# Autodesk Inventor assembly: illuminationAxis
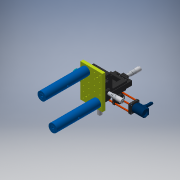
[picture p0: Inventor's stored thumbnail of the model, 180x180]
Saved by Autodesk Inventor 2016 (Build 200138000, 138)
## iProperties
Created: 2016-02-18
Part Number: illuminationAxis
Document SubType Name: Assembly
Designer: sims01
Author: sims01
## Documents named in this file (13)
- H:\Documents\LSFM_3\setup\mechanical\design\lsfm3_mechDesign\illuminationAxis.iam
- H:\Documents\LSFM_3\setup\mechanical\design\lsfm3_mechDesign\thorlabs100150mm2breadboard.ipt
- H:\Documents\LSFM_3\setup\mechanical\design\lsfm3_mechDesign\30mmCageMountingBase.ipt
- H:\Documents\LSFM_3\setup\mechanical\design\lsfm3_mechDesign\sm1CageMount.ipt
- H:\Documents\LSFM_3\setup\mechanical\design\lsfm3_mechDesign\m26sm1ThreadAdapter.ipt
- H:\Documents\LSFM_3\setup\mechanical\design\lsfm3_mechDesign\10X_mitutoyoObj.ipt
- H:\Documents\LSFM_3\setup\mechanical\design\lsfm3_mechDesign\30mmCageRotationMount.ipt
- H:\Documents\LSFM_3\setup\mechanical\design\lsfm3_mechDesign\75mmCylLens.ipt
- H:\Documents\LSFM_3\setup\mechanical\design\lsfm3_mechDesign\12mmFibreCollimator.ipt
- H:\Documents\LSFM_3\setup\mechanical\design\lsfm3_mechDesign\203mmCageRods.ipt
- H:\Documents\LSFM_3\setup\mechanical\design\lsfm3_mechDesign\graduatedIris.ipt
- H:\Documents\LSFM_3\setup\mechanical\design\lsfm3_mechDesign\translationStageAssembly.iam
- H:\Documents\LSFM_3\setup\mechanical\design\lsfm3_mechDesign\210mmPost.iam
## Components (20 placed, 12 different names)
1. thorlabs100150mm2breadboard:1 — Rigid:42, Rigid:48, Rigid:49
2. 30mmCageMountingBase:1 — Rigid:43, Rigid:46
3. sm1CageMount:1 — Rigid:31, Mate:25, Mate:26, Mate:27, Mate:28
4. m26sm1ThreadAdapter:1 — Rigid:7, Rigid:31
5. 10X_mitutoyoObj:1 — Rigid:7
6. 30mmCageRotationMount:1 — Rigid:47, Mate:29, Mate:30, Mate:31, Mate:32
7. 75mmCylLens:1 — Rigid:47
8. 12mmFibreCollimator:1 — Rigid:15
9. 203mmCageRods:1 — Mate:21, Mate:26, Mate:30, Mate:33
10. 203mmCageRods:2 — Mate:23, Mate:27, Mate:31, Mate:36
11. 203mmCageRods:3 — Mate:24, Mate:25, Mate:29, Mate:34
12. 203mmCageRods:4 — Mate:22, Mate:28, Mate:32, Mate:35
13. sm1CageMount:2 — Rigid:41, Rigid:45, Mate:21, Mate:22, Mate:23, Mate:24
14. sm1CageMount:3 — Rigid:15, Mate:33, Mate:34, Mate:35, Mate:36
15. sm1CageMount:4 — Rigid:46
16. 30mmCageMountingBase:2 — Rigid:44, Rigid:45
17. graduatedIris:1 — Rigid:41
18. translationStageAssembly:1 [sub-assembly] — Rigid:42, Rigid:43, Rigid:44
19. 210mmPost:1 [sub-assembly] — Rigid:49
20. 210mmPost:2 [sub-assembly] — Rigid:48
## Relationships (28: Mate 16, WeldJoint 12)
- Rigid:7 [WeldJoint] (-2.05 mm): m26sm1ThreadAdapter:1 ↔ 10X_mitutoyoObj:1
- Rigid:15 [WeldJoint]: 12mmFibreCollimator:1 ↔ sm1CageMount:3
- Rigid:31 [WeldJoint]: sm1CageMount:1 ↔ m26sm1ThreadAdapter:1
- Rigid:41 [WeldJoint]: sm1CageMount:2 ↔ graduatedIris:1
- Rigid:42 [WeldJoint]: thorlabs100150mm2breadboard:1 ↔ translationStageAssembly:1
- Rigid:43 [WeldJoint]: 30mmCageMountingBase:1 ↔ translationStageAssembly:1
- Rigid:44 [WeldJoint]: 30mmCageMountingBase:2 ↔ translationStageAssembly:1
- Rigid:45 [WeldJoint]: sm1CageMount:2 ↔ 30mmCageMountingBase:2
- Rigid:46 [WeldJoint]: 30mmCageMountingBase:1 ↔ sm1CageMount:4
- Mate:21: 203mmCageRods:1 ↔ sm1CageMount:2
- Mate:22: 203mmCageRods:4 ↔ sm1CageMount:2
- Mate:23: 203mmCageRods:2 ↔ sm1CageMount:2
- Mate:24: 203mmCageRods:3 ↔ sm1CageMount:2
- Mate:25: sm1CageMount:1 ↔ 203mmCageRods:3
- Mate:26: sm1CageMount:1 ↔ 203mmCageRods:1
- Mate:27: sm1CageMount:1 ↔ 203mmCageRods:2
- Mate:28: sm1CageMount:1 ↔ 203mmCageRods:4
- Rigid:47 [WeldJoint]: 30mmCageRotationMount:1 ↔ 75mmCylLens:1
- Mate:29: 30mmCageRotationMount:1 ↔ 203mmCageRods:3
- Mate:30: 30mmCageRotationMount:1 ↔ 203mmCageRods:1
- Mate:31: 30mmCageRotationMount:1 ↔ 203mmCageRods:2
- Mate:32: 30mmCageRotationMount:1 ↔ 203mmCageRods:4
- Mate:33: 203mmCageRods:1 ↔ sm1CageMount:3
- Mate:34: 203mmCageRods:3 ↔ sm1CageMount:3
- Mate:35: 203mmCageRods:4 ↔ sm1CageMount:3
- Mate:36: 203mmCageRods:2 ↔ sm1CageMount:3
- Rigid:48 [WeldJoint]: thorlabs100150mm2breadboard:1 ↔ 210mmPost:2
- Rigid:49 [WeldJoint]: thorlabs100150mm2breadboard:1 ↔ 210mmPost:1
